# Autodesk Inventor assembly: PumpingRegionNipple
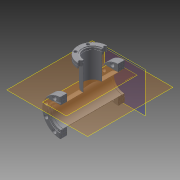
[picture p0: Inventor's stored thumbnail of the model, 180x180]
Saved by Autodesk Inventor 2015 (Build 190159000, 159)
## iProperties
Created: 2014-05-19
Part Number: PumpingRegionNipple
Document SubType Name: Assembly
Designer: jad211
Author: jad211
## Documents named in this file (4)
- C:\CADFiles\EDM Machine\EDM New Pumping Region\PumpingRegionNipple.iam
- C:\CADFiles\Generic vacuum components\3and38s Counter Bored.ipt
- C:\CADFiles\Generic vacuum components\DN35CF Counter Bored.ipt
- C:\CADFiles\EDM Machine\EDM New Pumping Region\51mm nipple.ipt
## Components (4 placed, 3 different names)
1. 3and38s Counter Bored:1 — Mate:1, Flush:1, Insert:2
2. DN35CF Counter Bored:1 — Insert:3
3. 3and38s Counter Bored:2 — Insert:1
4. 51mm nipple:1 — Insert:1, Insert:2, Insert:3
## Relationships (8: Mate 3, Insert 3, Flush 1, Angle 1)
- Mate:1: 3and38s Counter Bored:1
- Mate:2
- Flush:1: 3and38s Counter Bored:1
- Mate:3
- Angle:1 (0 deg)
- Insert:1: 3and38s Counter Bored:2 ↔ 51mm nipple:1
- Insert:2: 3and38s Counter Bored:1 ↔ 51mm nipple:1
- Insert:3: DN35CF Counter Bored:1 ↔ 51mm nipple:1
